# Autodesk Inventor assembly: Ensamble Mecanismo cilindro
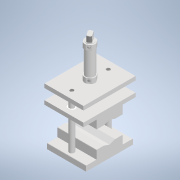
[picture p0: Inventor's stored thumbnail of the model, 180x180]
Saved by Autodesk Inventor 2021 (Build 250183000, 183)
## iProperties
Created: 2020-01-15
Part Number: Ensamble Mecanismo cilindro
Document SubType Name: Assembly
Designer: Nelson
Sending System: SolidWorks 2020
Last Author: Micro
Last Saved: 2020-01-16
Author: Nelson
## Documents named in this file (9)
- D:\Nelson\Documentos\Inventor\PrensaHidraulica_Automatizada\Ensamble Mecanismo cilindro.iam
- Ensamble mecanismo cilindro.iam
- D:\Nelson\Documentos\Inventor\PrensaHidraulica_Automatizada\Base soporte tubos.ipt
- D:\Nelson\Documentos\Inventor\PrensaHidraulica_Automatizada\Eje roscado base soporte tubo.ipt
- D:\Nelson\Documentos\Inventor\PrensaHidraulica_Automatizada\193992 DSNU-32-60-PPS-A---(60PPSA---00--0-------0).iam
- D:\Nelson\Documentos\Inventor\PrensaHidraulica_Automatizada\Soporte Piston.ipt
- D:\Nelson\Documentos\Inventor\PrensaHidraulica_Automatizada\Soporte Superior Tubos.ipt
- D:\Nelson\Documentos\Inventor\PrensaHidraulica_Automatizada\Buje soporte superior.ipt
- D:\Nelson\Documentos\Inventor\PrensaHidraulica_Automatizada\DIN 7984 - M8 x 20.ipt
## Components (12 placed, 7 different names)
1. Base soporte tubos:1 — Mate:27, Mate:28, Mate:30, Mate:47
2. Eje roscado base soporte tubo:1 — Mate:27, Mate:28, Mate:48, Mate:56, Mate:57
3. Eje roscado base soporte tubo:2 — Mate:30, Mate:47, Mate:49, Mate:58
4. Soporte Piston:1 — Mate:52, Mate:53, Mate:56, Mate:57, Mate:58, Mate:59, Mate:60, Flush:1, Flush:2
5. Soporte Superior Tubos:1 — Mate:36, Mate:37, Mate:38, Mate:39, Mate:40, Mate:41, Mate:42, Mate:43, Mate:50, Mate:51
6. Buje soporte superior:1 — Mate:38, Mate:39, Mate:49
7. Buje soporte superior:2 — Mate:36, Mate:37, Mate:48
8. Buje soporte superior:3 — Mate:40, Mate:41
9. Buje soporte superior:4 — Mate:42, Mate:43
10. 193992 DSNU-32-60-PPS-A---(60PPSA---00--0-------0):1 [sub-assembly] — Mate:50, Mate:51, Mate:52, Mate:53
11. DIN 7984 M8 x 20:1 — Mate:59, Flush:1
12. DIN 7984 M8 x 20:2 — Mate:60, Flush:2
## Relationships (25: Mate 23, Flush 2)
- Mate:27: Base soporte tubos:1 ↔ Eje roscado base soporte tubo:1
- Mate:28: Base soporte tubos:1 ↔ Eje roscado base soporte tubo:1
- Mate:30: Base soporte tubos:1 ↔ Eje roscado base soporte tubo:2
- Mate:36: Soporte Superior Tubos:1 ↔ Buje soporte superior:2
- Mate:37: Soporte Superior Tubos:1 ↔ Buje soporte superior:2
- Mate:38: Soporte Superior Tubos:1 ↔ Buje soporte superior:1
- Mate:39: Soporte Superior Tubos:1 ↔ Buje soporte superior:1
- Mate:40: Soporte Superior Tubos:1 ↔ Buje soporte superior:3
- Mate:41: Soporte Superior Tubos:1 ↔ Buje soporte superior:3
- Mate:42: Soporte Superior Tubos:1 ↔ Buje soporte superior:4
- Mate:43: Soporte Superior Tubos:1 ↔ Buje soporte superior:4
- Mate:47: Base soporte tubos:1 ↔ Eje roscado base soporte tubo:2
- Mate:48: Eje roscado base soporte tubo:1 ↔ Buje soporte superior:2
- Mate:49: Eje roscado base soporte tubo:2 ↔ Buje soporte superior:1
- Mate:50: Soporte Superior Tubos:1 ↔ 193992 DSNU-32-60-PPS-A---(60PPSA---00--0-------0):1
- Mate:51: Soporte Superior Tubos:1 ↔ 193992 DSNU-32-60-PPS-A---(60PPSA---00--0-------0):1
- Mate:52: Soporte Piston:1 ↔ 193992 DSNU-32-60-PPS-A---(60PPSA---00--0-------0):1
- Mate:53: Soporte Piston:1 ↔ 193992 DSNU-32-60-PPS-A---(60PPSA---00--0-------0):1
- Mate:56: Eje roscado base soporte tubo:1 ↔ Soporte Piston:1
- Mate:57: Eje roscado base soporte tubo:1 ↔ Soporte Piston:1
- Mate:58: Eje roscado base soporte tubo:2 ↔ Soporte Piston:1
- Mate:59: Soporte Piston:1 ↔ DIN 7984 M8 x 20:1
- Mate:60: Soporte Piston:1 ↔ DIN 7984 M8 x 20:2
- Flush:1: Soporte Piston:1 ↔ DIN 7984 M8 x 20:1
- Flush:2: Soporte Piston:1 ↔ DIN 7984 M8 x 20:2
